# Autodesk Inventor assembly: Dribbler
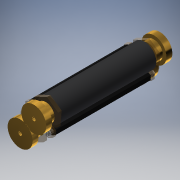
[picture p0: Inventor's stored thumbnail of the model, 180x180]
Saved by Autodesk Inventor 2017 (Build 210142000, 142)
## iProperties
Created: 2017-04-14
Part Number: Dribbler
Document SubType Name: Assembly
Designer: yella
Author: yella
## Documents named in this file (7)
- C:\Users\yella\git\LJ-STAND\Design\Models\Robot\Dribbler.iam
- C:\Users\yella\git\LJ-STAND\Design\Models\Robot\Dribbler Barrel.ipt
- C:\Users\yella\git\LJ-STAND\Design\Models\Robot\Dribbler Plate.ipt
- C:\Users\yella\git\LJ-STAND\Design\Models\Common\micro-metal-gearmotor-carbon.ipt
- C:\Users\yella\git\LJ-STAND\Design\Models\Common\Gear.ipt
- C:\Users\yella\git\LJ-STAND\Design\Models\Fasteners\M3x10 Screw.ipt
- C:\Users\yella\git\LJ-STAND\Design\Models\Fasteners\Standoff 80 F-F.ipt
## Components (15 placed, 6 different names)
1. Gear:1 — Insert:12
2. Gear:2 — Insert:13
3. Gear:3 — Insert:7
4. Gear:4 — Insert:6
5. micro-metal-gearmotor-carbon:1 — Insert:3, Insert:11
6. micro-metal-gearmotor-carbon:2 — Insert:1, Insert:2
7. Dribbler Plate:1 — Insert:1, Insert:2, Insert:4, Insert:5, Insert:6, Insert:7, Insert:8, Insert:16, Insert:17
8. Dribbler Plate:2 — Insert:3, Insert:9, Insert:10, Insert:11, Insert:12, Insert:13, Insert:14, Insert:15
9. M3x10 Screw:1 — Insert:15
10. M3x10 Screw:2 — Insert:16
11. M3x10 Screw:3 — Insert:14
12. M3x10 Screw:4 — Insert:17
13. Standoff 80 F-F:1 — Insert:4, Insert:9
14. Standoff 80 F-F:2 — Insert:5, Insert:10
15. Dribbler Barrel:1 — Insert:8
## Relationships (17: Insert 17)
- Insert:1: micro-metal-gearmotor-carbon:2 ↔ Dribbler Plate:1
- Insert:2: micro-metal-gearmotor-carbon:2 ↔ Dribbler Plate:1
- Insert:3: micro-metal-gearmotor-carbon:1 ↔ Dribbler Plate:2
- Insert:4: Dribbler Plate:1 ↔ Standoff 80 F-F:1
- Insert:5: Dribbler Plate:1 ↔ Standoff 80 F-F:2
- Insert:6: Gear:4 ↔ Dribbler Plate:1
- Insert:7: Gear:3 ↔ Dribbler Plate:1
- Insert:8: Dribbler Plate:1 ↔ Dribbler Barrel:1
- Insert:9: Dribbler Plate:2 ↔ Standoff 80 F-F:1
- Insert:10: Dribbler Plate:2 ↔ Standoff 80 F-F:2
- Insert:11: micro-metal-gearmotor-carbon:1 ↔ Dribbler Plate:2
- Insert:12: Gear:1 ↔ Dribbler Plate:2
- Insert:13: Gear:2 ↔ Dribbler Plate:2
- Insert:14: Dribbler Plate:2 ↔ M3x10 Screw:3
- Insert:15: Dribbler Plate:2 ↔ M3x10 Screw:1
- Insert:16: Dribbler Plate:1 ↔ M3x10 Screw:2
- Insert:17: Dribbler Plate:1 ↔ M3x10 Screw:4
